# Autodesk Inventor assembly: Receptor (Trilho inferior)
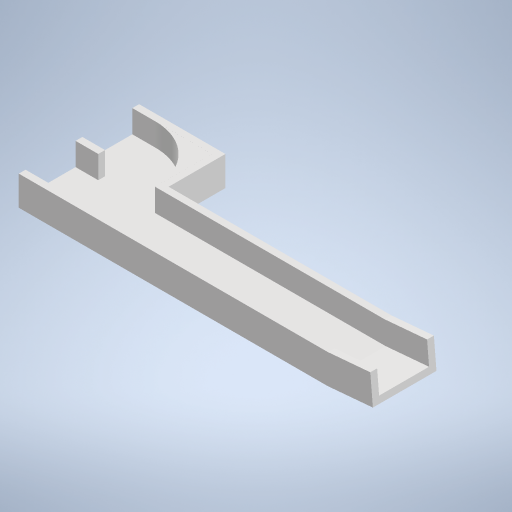
[picture p0: Inventor's stored thumbnail of the model, 512x512]
Saved by Autodesk Inventor 2024 (Build 280153020, 153B)
## iProperties
Created: 2023-05-29
Part Number: Receptor (Trilho inferior)
Document SubType Name: Assembly
Designer: jpjoa
Author: jpjoa
## Documents named in this file (3)
- G:\.shortcut-targets-by-id\1lOMf-Kp8UroJbDMtxyO7ak_I_KYCWiat\Faculdade\Trabalhos\Desenho e Print 3D\Marbles 2.0\Peças montadas\Receptor (Trilho inferior).iam
- G:\.shortcut-targets-by-id\1lOMf-Kp8UroJbDMtxyO7ak_I_KYCWiat\Faculdade\Trabalhos\Desenho e Print 3D\Marbles 2.0\Trilho receptor (inferior).ipt
- G:\.shortcut-targets-by-id\1lOMf-Kp8UroJbDMtxyO7ak_I_KYCWiat\Faculdade\Trabalhos\Desenho e Print 3D\Marbles 2.0\Encaixe (trilhos).ipt
## Components (2 placed, 2 different names)
1. Trilho receptor (inferior):1 — Coincidente:1, Coincidente:2, Coincidente:3
2. Encaixe (trilhos):1 — Coincidente:1, Coincidente:2, Coincidente:3
## Relationships (3: Mate 3)
- Coincidente:1 [Mate]: Trilho receptor (inferior):1 ↔ Encaixe (trilhos):1
- Coincidente:2 [Mate]: Trilho receptor (inferior):1 ↔ Encaixe (trilhos):1
- Coincidente:3 [Mate]: Trilho receptor (inferior):1 ↔ Encaixe (trilhos):1
